# Autodesk Inventor assembly: DribblerUnit
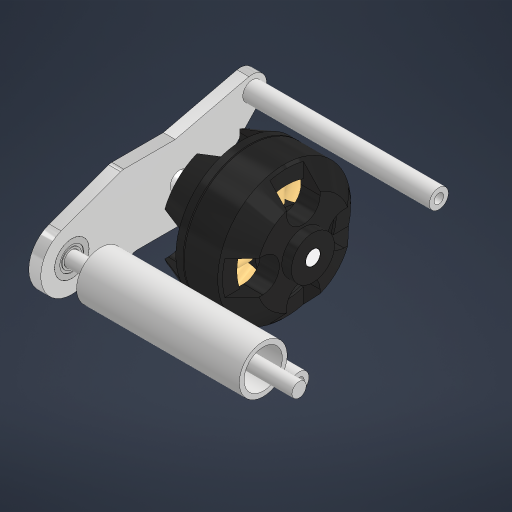
[picture p0: Inventor's stored thumbnail of the model, 512x512]
Saved by Autodesk Inventor 2024.2 (Build 282272000, 272)
## iProperties
Created: 2023-12-27
Part Number: DribblerUnit
Document SubType Name: Assembly
Designer: Hanaoka
Author: Hanaoka
## Documents named in this file (7)
- G:\共有ドライブ\reRo\05_個人\hanaoka\inventor\DribblerUnit\DribblerUnit.iam
- G:\共有ドライブ\reRo\05_個人\hanaoka\inventor\HandleUnit\GearCover.ipt
- G:\共有ドライブ\reRo\05_個人\hanaoka\inventor\DribblerUnit\Shaft.ipt
- G:\共有ドライブ\reRo\05_個人\hanaoka\inventor\DribblerUnit\Bearing_C-FL673ZZ.ipt
- G:\共有ドライブ\reRo\05_個人\hanaoka\inventor\DribblerUnit\tube.ipt
- G:\共有ドライブ\reRo\05_個人\hanaoka\inventor\DribblerUnit\SHaft_m2x40.ipt
- G:\共有ドライブ\reRo\05_個人\hanaoka\inventor\DribblerUnit\C2822 1400KV BLDC v25\C2822 1400KV BLDC v25.ipt
## Components (7 placed, 6 different names)
1. GearCover:1 — 挿入:1, 挿入:7, 挿入:9, 挿入:10
2. Shaft:1 — 挿入:2
3. Bearing_C-FL673ZZ:1 — 挿入:1, 挿入:2
4. tube:1 — 挿入:9
5. SHaft_m2x40:1 — 挿入:7
6. C2822 1400KV BLDC v25:1
7. SHaft_m2x40:2 — 挿入:10
## Relationships (5: Insert 5)
- 挿入:1 [Insert]: GearCover:1 ↔ Bearing_C-FL673ZZ:1
- 挿入:2 [Insert]: Shaft:1 ↔ Bearing_C-FL673ZZ:1
- 挿入:7 [Insert]: GearCover:1 ↔ SHaft_m2x40:1
- 挿入:9 [Insert] (6 mm): GearCover:1 ↔ tube:1
- 挿入:10 [Insert]: GearCover:1 ↔ SHaft_m2x40:2
